# Autodesk Inventor assembly: ASY TZS 1752 FDS way 2
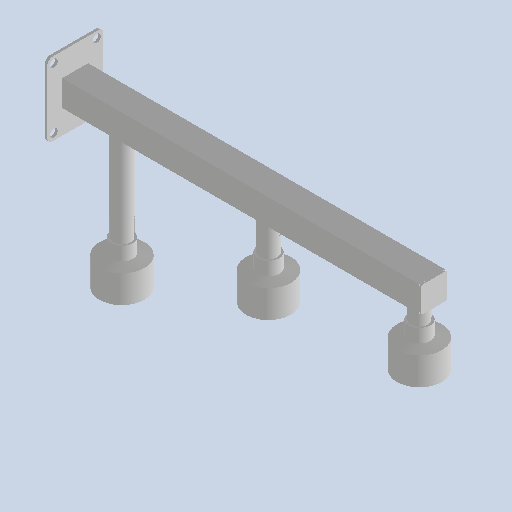
[picture p0: Inventor's stored thumbnail of the model, 512x512]
Saved by Autodesk Inventor 2025 (Build 290162010, 162A)
## iProperties
Created: 2025-07-02
Part Number: ASY TZS 1752 FDS way 2
Document SubType Name: Assembly
Designer: user
Author: user
## Documents named in this file (8)
- C:\Users\pokla\Documents\Inventor\TZS-Tazovskiy\Filter D1200\FDS\ASY TZS 1752 FDS way 2.iam
- C:\Users\pokla\Documents\Inventor\TZS-Tazovskiy\Filter D1200\FDS\TZS 1752 FDS 1200 way tube 2.ipt
- C:\Users\pokla\Documents\Inventor\TZS-Tazovskiy\Filter D1200\FDS\TZS dummy filter element.ipt
- C:\Users\pokla\Documents\Inventor\TZS-Tazovskiy\Filter D1200\FDS\TZS dummy pipe nippel.ipt
- C:\Users\pokla\Documents\Inventor\TZS-Tazovskiy\Filter D1200\FDS\TZS 1756 FDS 1200 way tube 6.ipt
- C:\Users\pokla\Documents\Inventor\TZS-Tazovskiy\Filter D1200\FDS\TZS 1757 FDS 1200 way tube 7.ipt
- C:\Users\pokla\Documents\Inventor\TZS-Tazovskiy\Filter D1200\FDS\TZS 760 FDS 1200 FLANGE 3.ipt
- C:\Users\pokla\Documents\Inventor\TZS-Tazovskiy\Filter D1200\FDS\TZS 766 FDS 1200 CUP 1.ipt
## Components (11 placed, 7 different names)
1. TZS 1752 FDS 1200 way tube 2.ipt:1
2. TZS dummy filter element.ipt:1
3. TZS dummy pipe nippel.ipt:1
4. TZS 1756 FDS 1200 way tube 6.ipt:1
5. TZS dummy filter element.ipt:2
6. TZS dummy pipe nippel.ipt:2
7. TZS 1757 FDS 1200 way tube 7.ipt:1
8. TZS dummy filter element.ipt:3
9. TZS dummy pipe nippel.ipt:3
10. TZS 760 FDS 1200 FLANGE 3.ipt:1
11. TZS 766 FDS 1200 CUP 1.ipt:1
## Relationships (10: WeldJoint 10)
- [WeldJoint]: TZS dummy filter element.ipt:1 ↔ TZS dummy pipe nippel.ipt:1
- [WeldJoint]: TZS 1752 FDS 1200 way tube 2.ipt:1 ↔ TZS dummy pipe nippel.ipt:1
- [WeldJoint]: TZS dummy filter element.ipt:2 ↔ TZS dummy pipe nippel.ipt:2
- [WeldJoint]: TZS 1756 FDS 1200 way tube 6.ipt:1 ↔ TZS dummy pipe nippel.ipt:2
- [WeldJoint]: TZS 1752 FDS 1200 way tube 2.ipt:1 ↔ TZS 1756 FDS 1200 way tube 6.ipt:1
- [WeldJoint]: TZS dummy filter element.ipt:3 ↔ TZS dummy pipe nippel.ipt:3
- [WeldJoint]: TZS 1757 FDS 1200 way tube 7.ipt:1 ↔ TZS dummy pipe nippel.ipt:3
- [WeldJoint]: TZS 1752 FDS 1200 way tube 2.ipt:1 ↔ TZS 1757 FDS 1200 way tube 7.ipt:1
- [WeldJoint] (-3 mm): TZS 1752 FDS 1200 way tube 2.ipt:1 ↔ TZS 760 FDS 1200 FLANGE 3.ipt:1
- [WeldJoint]: TZS 1752 FDS 1200 way tube 2.ipt:1 ↔ TZS 766 FDS 1200 CUP 1.ipt:1
## Named parameters: d40_d37_d34_d31 = 0 mm, d49_d45_d43_d40_d37_d34_d31 = 0 mm, d50_d46 = 0 mm
